# Autodesk Inventor assembly: First Extension of Base
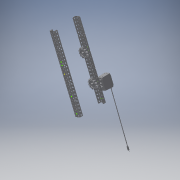
[picture p0: Inventor's stored thumbnail of the model, 180x180]
Saved by Autodesk Inventor 2018 (Build 220112000, 112)
## iProperties
Created: 2017-06-28
Part Number: First Extension of Base
Document SubType Name: Assembly
Designer: James
Author: James
## Documents named in this file (4)
- C:\Users\James\Desktop\EE REU\Hardware\Vex Arm\First Extension of Base.iam
- C:\Users\James\Desktop\EE REU\Hardware\Vex Arm\Vex Parts\C_Channel.ipt
- C:\Users\James\Desktop\EE REU\Hardware\Vex Arm\Vex Parts\Vex Sprocket Kit\sprocket-hs-12-tooth.ipt
- C:\Users\James\Desktop\EE REU\Hardware\Vex Arm\Vex Parts\393motor.ipt
## Components (5 placed, 3 different names)
1. C_Channel:1 — Flush:1, Mate:1, Flush:2
2. C_Channel:2 — Flush:1, Mate:1, Flush:2, Insert:1, Insert:2, Insert:3
3. sprocket-hs-12-tooth:1 — Insert:1
4. sprocket-hs-12-tooth:2 — Insert:2
5. 393motor:1 — Insert:3
## Relationships (6: Insert 3, Flush 2, Mate 1)
- Flush:1: C_Channel:1 ↔ C_Channel:2
- Mate:1 (120 mm): C_Channel:1 ↔ C_Channel:2
- Flush:2: C_Channel:1 ↔ C_Channel:2
- Insert:1 (20 mm): C_Channel:2 ↔ sprocket-hs-12-tooth:1
- Insert:2 (20 mm): C_Channel:2 ↔ sprocket-hs-12-tooth:2
- Insert:3 (20 mm): C_Channel:2 ↔ 393motor:1
